# Autodesk Inventor assembly: ЛЦМК0000002.00.00.00.00.10
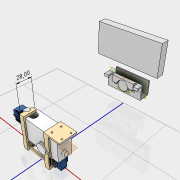
[picture p0: Inventor's stored thumbnail of the model, 180x180]
Saved by Autodesk Inventor 2021.2 (Build 252289000, 289)
## iProperties
Created: 2025-10-23
Part Number: ЛЦМК0000002.00.00.00.00.10
Document SubType Name: Assembly
Designer: Захаров
Author: Захаров
## Documents named in this file (9)
- C:\Users\User\Documents\ARHeadGen1\ЛЦМК0000002.00.00.00.00.10.iam
- C:\Users\User\Documents\ARHeadGen1\ЛЦМК0000002.00.00.00.00.05.ipt
- C:\Users\User\Documents\ARHeadGen1\Сборка1.iam
- C:\Users\User\Documents\ARHeadGen1\ЛЦМК000002.00.00.00.00.02.ipt
- C:\Users\User\Documents\ARHeadGen1\ЛЦМК000002.00.00.00.00.07.ipt
- C:\Users\User\Documents\ARHeadGen1\ЛЦМК000002.00.00.00.00.08.ipt
- C:\Users\User\Documents\ARHeadGen1\ЛЦМК000002.00.00.00.00.09.ipt
- C:\Users\User\Documents\ARHeadGen1\ЛЦМК000002.00.00.00.00.10.ipt
- C:\Users\User\Documents\ARHeadGen1\ЛЦМК000002.00.00.00.00.06-02.ipt
## Components (9 placed, 8 different names)
1. ЛЦМК0000002.00.00.00.00.05:1 — Заподлицо:8
2. Сборка1:1 [sub-assembly]
3. Сборка1:2 [sub-assembly] — Flush:7
4. ЛЦМК000002.00.00.00.00.06-02:1
5. ЛЦМК000002.00.00.00.00.02:1
6. ЛЦМК000002.00.00.00.00.07:1 — Flush:7
7. ЛЦМК000002.00.00.00.00.08:1 — Заподлицо:8, Заподлицо:9
8. ЛЦМК000002.00.00.00.00.09:1 — Заподлицо:9, Заподлицо:10
9. ЛЦМК000002.00.00.00.00.10:1 — Заподлицо:10
## Relationships (4: Flush 4)
- Flush:7: Сборка1:2 ↔ ЛЦМК000002.00.00.00.00.07:1
- Заподлицо:8 [Flush] (180 mm): ЛЦМК0000002.00.00.00.00.05:1 ↔ ЛЦМК000002.00.00.00.00.08:1
- Заподлицо:9 [Flush]: ЛЦМК000002.00.00.00.00.08:1 ↔ ЛЦМК000002.00.00.00.00.09:1
- Заподлицо:10 [Flush]: ЛЦМК000002.00.00.00.00.09:1 ↔ ЛЦМК000002.00.00.00.00.10:1
